# Autodesk Inventor assembly: X_Führung
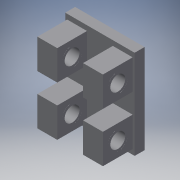
[picture p0: Inventor's stored thumbnail of the model, 180x180]
Saved by Autodesk Inventor 2019 (Build 230136000, 136)
## iProperties
Created: 2018-08-19
Part Number: X_Führung
Document SubType Name: Assembly
Designer: Julia
Author: Julia
## Documents named in this file (3)
- C:\Users\Julia\Documents\Inventor\3D_Drucker_v01\X_Führung.iam
- C:\Users\Julia\Documents\Inventor\3D_Drucker_v01\Y_Slider.ipt
- C:\Users\Julia\Documents\Inventor\3D_Drucker_v01\Metallstange_Slider.ipt
## Components (5 placed, 2 different names)
1. Y_Slider:1 — Insert:1, Insert:2, Insert:3, Insert:4
2. Metallstange_Slider:1 — Insert:1
3. Metallstange_Slider:2 — Insert:2
4. Metallstange_Slider:3 — Insert:3
5. Metallstange_Slider:4 — Insert:4
## Relationships (4: Insert 4)
- Insert:1: Y_Slider:1 ↔ Metallstange_Slider:1
- Insert:2: Y_Slider:1 ↔ Metallstange_Slider:2
- Insert:3: Y_Slider:1 ↔ Metallstange_Slider:3
- Insert:4: Y_Slider:1 ↔ Metallstange_Slider:4
